# Autodesk Inventor assembly: Assembly1
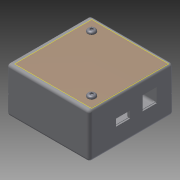
[picture p0: Inventor's stored thumbnail of the model, 180x180]
Saved by Autodesk Inventor 2013 (Build 170138000, 138)
## iProperties
Created: 2013-01-09
Part Number: Assembly1
Document SubType Name: Assembly
Designer: md
Author: md
## Documents named in this file (5)
- X:\Projects\hexasense\enclosure\Assembly1.iam
- X:\Projects\hexasense\enclosure\Unterschale.ipt
- C:\Users\md\Documents\Inventor\Content Center Files\R2013\en-US\ANSI B 18.2.4.1 M(1)\ANSI B 18.2.4.1 M - M3 x 0,5Style 1.ipt
- X:\Projects\hexasense\enclosure\Oberschale.ipt
- C:\Users\md\Documents\Inventor\Content Center Files\R2013\en-US\ANSI B18.3.4M(1)\ANSI B18.3.4M - M3 x 0.5 x 35(2).ipt
## Components (6 placed, 4 different names)
1. Unterschale:1 — Flush:1, Mate:3, Mate:4, Flush:2, Mate:5, Mate:6, Mate:7
2. Hex Nut Metric M3 x 0,5:1 — Flush:1, Mate:4
3. Hex Nut Metric M3 x 0,5:2 — Mate:3, Flush:2
4. Oberschale:1 — Mate:5, Mate:6, Mate:7, Mate:8, Mate:9, Mate:10, Mate:11
5. Broached Hexagon Socket Button Head Cap Screw - Metric M3 x 0.5 x 35:1 — Mate:8, Mate:9
6. Broached Hexagon Socket Button Head Cap Screw - Metric M3 x 0.5 x 35:2 — Mate:10, Mate:11
## Relationships (11: Mate 9, Flush 2)
- Flush:1: Unterschale:1 ↔ Hex Nut Metric M3 x 0,5:1
- Mate:3: Unterschale:1 ↔ Hex Nut Metric M3 x 0,5:2
- Mate:4: Unterschale:1 ↔ Hex Nut Metric M3 x 0,5:1
- Flush:2: Unterschale:1 ↔ Hex Nut Metric M3 x 0,5:2
- Mate:5: Unterschale:1 ↔ Oberschale:1
- Mate:6: Unterschale:1 ↔ Oberschale:1
- Mate:7: Unterschale:1 ↔ Oberschale:1
- Mate:9: Oberschale:1 ↔ Broached Hexagon Socket Button Head Cap Screw - Metric M3 x 0.5 x 35:1
- Mate:11: Oberschale:1 ↔ Broached Hexagon Socket Button Head Cap Screw - Metric M3 x 0.5 x 35:2
- Mate:8: Oberschale:1 ↔ Broached Hexagon Socket Button Head Cap Screw - Metric M3 x 0.5 x 35:1
- Mate:10: Oberschale:1 ↔ Broached Hexagon Socket Button Head Cap Screw - Metric M3 x 0.5 x 35:2
